# Autodesk Inventor assembly: Button box assembly
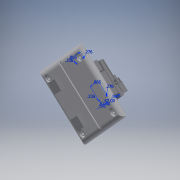
[picture p0: Inventor's stored thumbnail of the model, 180x180]
Saved by Autodesk Inventor 2018 (Build 220112000, 112)
## iProperties
Created: 2019-09-19
Part Number: Button box assembly
Document SubType Name: Assembly
Designer: Jacob
Author: Jacob
## Documents named in this file (11)
- C:\Users\Jacob\git_repos\POE-CAD\Fall 2019 Cad Files\CAD Files\Button box assembly.iam
- C:\Users\Jacob\git_repos\POE-CAD\Fall 2019 Cad Files\CAD Files\RFID Card Reader.ipt
- C:\Users\Jacob\git_repos\POE-CAD\Fall 2019 Cad Files\CAD Files\2 gang light switch plate.ipt
- C:\Users\Jacob\git_repos\POE-CAD\Fall 2019 Cad Files\CAD Files\POE splitter.ipt
- C:\Users\Jacob\git_repos\POE-CAD\Fall 2019 Cad Files\CAD Files\Official parts\RaspberryPiZeroW.ipt
- C:\Users\Jacob\git_repos\POE-CAD\Fall 2019 Cad Files\CAD Files\Button.ipt
- C:\Users\Jacob\git_repos\POE-AIO\CAD Files\PI Rfid baracke angledt.ipt
- C:\Users\Jacob\git_repos\POE-CAD\Fall 2019 Cad Files\CAD Files\New Parts\POE line bracket.ipt
- C:\Users\Jacob\git_repos\POE-CAD\Fall 2019 Cad Files\CAD Files\New Parts\Final smaller ethernet.ipt
- C:\Users\Jacob\git_repos\POE-CAD\Fall 2019 Cad Files\CAD Files\New Parts\New poe ethernet splitter holder.ipt
- C:\Users\Jacob\git_repos\POE-CAD\Fall 2019 Cad Files\CAD Files\New Parts\PI Rfid baracke angled reconfig.ipt
## Components (11 placed, 10 different names)
1. RFID Card Reader:1 — Mate:19, Mate:20, Mate:21, Mate:22, Mate:23, Mate:24, Mate:25, Mate:26, Mate:27
2. 2 gang light switch plate:1 — Mate:3, Mate:5, Mate:16, Mate:17, Mate:19, Mate:20, Mate:21
3. POE splitter:1 — Mate:30, Mate:31, Flush:1
4. RaspberryPiZeroW:1 — Mate:40, Mate:41
5. Button:1 — Mate:3, Mate:17
6. Button:2 — Mate:5, Mate:16
7. PI Rfid baracke angledt:1 — Mate:22, Mate:23, Mate:24
8. POE line bracket:1 — Mate:32, Mate:33, Mate:34, Mate:35
9. Final smaller ethernet:1 — Mate:34, Mate:35, Flush:2, Mate:36
10. New poe ethernet splitter holder:1 — Mate:30, Mate:31, Flush:1, Mate:32, Mate:33, Flush:2, Mate:36, Mate:42
11. PI Rfid baracke angled reconfig:1 — Mate:25, Mate:26, Mate:27, Mate:40, Mate:41, Mate:42
## Relationships (25: Mate 23, Flush 2)
- Mate:3: 2 gang light switch plate:1 ↔ Button:1
- Mate:5: 2 gang light switch plate:1 ↔ Button:2
- Mate:16: 2 gang light switch plate:1 ↔ Button:2
- Mate:17: 2 gang light switch plate:1 ↔ Button:1
- Mate:19: RFID Card Reader:1 ↔ 2 gang light switch plate:1
- Mate:20: RFID Card Reader:1 ↔ 2 gang light switch plate:1
- Mate:21: RFID Card Reader:1 ↔ 2 gang light switch plate:1
- Mate:22: RFID Card Reader:1 ↔ PI Rfid baracke angledt:1
- Mate:23: RFID Card Reader:1 ↔ PI Rfid baracke angledt:1
- Mate:24: RFID Card Reader:1 ↔ PI Rfid baracke angledt:1
- Mate:25: RFID Card Reader:1 ↔ PI Rfid baracke angled reconfig:1
- Mate:26: RFID Card Reader:1 ↔ PI Rfid baracke angled reconfig:1
- Mate:27: RFID Card Reader:1 ↔ PI Rfid baracke angled reconfig:1
- Mate:30: POE splitter:1 ↔ New poe ethernet splitter holder:1
- Mate:31: POE splitter:1 ↔ New poe ethernet splitter holder:1
- Flush:1: POE splitter:1 ↔ New poe ethernet splitter holder:1
- Mate:32: POE line bracket:1 ↔ New poe ethernet splitter holder:1
- Mate:33: POE line bracket:1 ↔ New poe ethernet splitter holder:1
- Mate:34: POE line bracket:1 ↔ Final smaller ethernet:1
- Mate:35: POE line bracket:1 ↔ Final smaller ethernet:1
- Flush:2: Final smaller ethernet:1 ↔ New poe ethernet splitter holder:1
- Mate:36: Final smaller ethernet:1 ↔ New poe ethernet splitter holder:1
- Mate:40: RaspberryPiZeroW:1 ↔ PI Rfid baracke angled reconfig:1
- Mate:41: RaspberryPiZeroW:1 ↔ PI Rfid baracke angled reconfig:1
- Mate:42: New poe ethernet splitter holder:1 ↔ PI Rfid baracke angled reconfig:1
